# Autodesk Inventor assembly: hipjoint
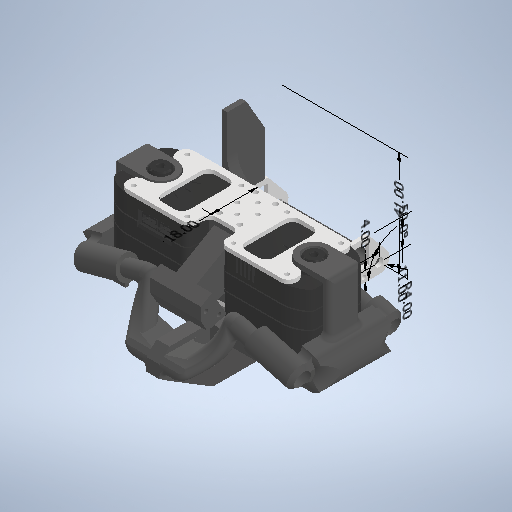
[picture p0: Inventor's stored thumbnail of the model, 512x512]
Saved by Autodesk Inventor 2026.1 (Build 301233020, 233B)
## iProperties
Created: 2024-10-09
Part Number: hipjoint
Document SubType Name: Assembly
Designer: hibik
Author: hibik
## Documents named in this file (9)
- C:\Users\hibik\Documents\Robomech\HR\Eglantyne_mark2\hard\under_body\hipjoint.iam
- C:\Users\hibik\Documents\Robomech\HR\Eglantyne_mark2\hard\under_body\hipjoint_upper.ipt
- C:\Users\hibik\Documents\Robomech\HR\Eglantyne_mark2\hard\needed_model\KRS3300モータ.ipt
- C:\Users\hibik\Documents\Robomech\HR\Eglantyne_mark2\hard\needed_model\KRS3300サーボホーン.ipt
- C:\Users\hibik\Documents\Robomech\HR\Eglantyne_mark2\hard\under_body\hipjoint_middle.ipt
- C:\Users\hibik\Documents\Robomech\HR\Eglantyne_mark2\hard\under_body\joit_cover_hip.ipt
- C:\Users\hibik\Documents\Robomech\HR\Eglantyne_mark2\hard\under_body\battery_cover_setter_joint.ipt
- C:\Users\hibik\Documents\Robomech\HR\Eglantyne_mark2\hard\under_body\joit_cover_hip_side.ipt
- C:\Users\hibik\Documents\Robomech\HR\Eglantyne_mark2\hard\under_body\joit_cover_hip_side_left.ipt
## Components (12 placed, 8 different names)
1. hipjoint_upper:1 — 挿入:1, 挿入:2, 角度:2, メイト:1, フラッシュ:1, メイト:2
2. KRS3300モータ:1 — 挿入:1, 角度:1, 挿入:3, 挿入:5, 挿入:6
3. KRS3300モータ:2 — 挿入:2, 角度:1, 角度:2, 挿入:4, メイト:5, 挿入:9
4. KRS3300サーボホーン:1 — 挿入:4
5. KRS3300サーボホーン:2 — 挿入:3
6. hipjoint_middle:1 — メイト:1, フラッシュ:1, メイト:2, フラッシュ:6, フラッシュ:7, メイト:6, メイト:7, フラッシュ:8, フラッシュ:9
7. hipjoint_upper:2 — メイト:5, 挿入:5, 挿入:6, 挿入:7, 挿入:8
8. joit_cover_hip:1 — 挿入:7, 挿入:8, フラッシュ:10, フラッシュ:11
9. battery_cover_setter_joint:1 — フラッシュ:6, フラッシュ:7, メイト:6
10. battery_cover_setter_joint:2 — メイト:7, フラッシュ:8, フラッシュ:9
11. joit_cover_hip_side:1 — 角度:3, フラッシュ:10, フラッシュ:11
12. joit_cover_hip_side_left:1 — 挿入:9
## Relationships (24: Insert 9, Flush 7, Mate 5, Angle 3)
- 挿入:1 [Insert]: hipjoint_upper:1 ↔ KRS3300モータ:1
- 挿入:2 [Insert]: hipjoint_upper:1 ↔ KRS3300モータ:2
- 角度:1 [Angle] (180 deg): KRS3300モータ:1 ↔ KRS3300モータ:2
- 角度:2 [Angle] (0 deg): hipjoint_upper:1 ↔ KRS3300モータ:2
- 挿入:3 [Insert]: KRS3300モータ:1 ↔ KRS3300サーボホーン:2
- 挿入:4 [Insert]: KRS3300モータ:2 ↔ KRS3300サーボホーン:1
- メイト:1 [Mate]: hipjoint_upper:1 ↔ hipjoint_middle:1
- フラッシュ:1 [Flush]: hipjoint_upper:1 ↔ hipjoint_middle:1
- メイト:2 [Mate]: hipjoint_upper:1 ↔ hipjoint_middle:1
- メイト:5 [Mate]: KRS3300モータ:2 ↔ hipjoint_upper:2
- 挿入:5 [Insert]: KRS3300モータ:1 ↔ hipjoint_upper:2
- 挿入:6 [Insert]: KRS3300モータ:1 ↔ hipjoint_upper:2
- 挿入:7 [Insert]: hipjoint_upper:2 ↔ joit_cover_hip:1
- 挿入:8 [Insert]: hipjoint_upper:2 ↔ joit_cover_hip:1
- フラッシュ:6 [Flush]: hipjoint_middle:1 ↔ battery_cover_setter_joint:1
- フラッシュ:7 [Flush]: hipjoint_middle:1 ↔ battery_cover_setter_joint:1
- メイト:6 [Mate]: hipjoint_middle:1 ↔ battery_cover_setter_joint:1
- メイト:7 [Mate]: hipjoint_middle:1 ↔ battery_cover_setter_joint:2
- フラッシュ:8 [Flush]: hipjoint_middle:1 ↔ battery_cover_setter_joint:2
- フラッシュ:9 [Flush]: hipjoint_middle:1 ↔ battery_cover_setter_joint:2
- 角度:3 [Angle] (0 deg): joit_cover_hip_side:1
- フラッシュ:10 [Flush]: joit_cover_hip:1 ↔ joit_cover_hip_side:1
- フラッシュ:11 [Flush]: joit_cover_hip:1 ↔ joit_cover_hip_side:1
- 挿入:9 [Insert]: KRS3300モータ:2 ↔ joit_cover_hip_side_left:1
